# Autodesk Inventor assembly: Spool mount
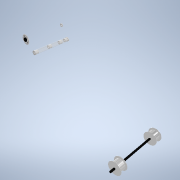
[picture p0: Inventor's stored thumbnail of the model, 180x180]
Saved by Autodesk Inventor 2020 (Build 240168000, 168)
## iProperties
Created: 2020-01-30
Part Number: Spool mount
Document SubType Name: Assembly
Designer: 1cikaychapman
Author: 1cikaychapman
## Documents named in this file (9)
- D:\Users\JimAndVal\Documents\JIM\IronRiders\2020 Robot-1\Climber\Spool mount.iam
- D:\Users\JimAndVal\Documents\JIM\IronRiders\2020 Robot-1\Climber\Hex.ipt
- D:\Users\JimAndVal\Documents\JIM\IronRiders\2020 Robot-1\Climber\Spool.ipt
- D:\Users\JimAndVal\Documents\JIM\IronRiders\2020 Robot-1\Climber\Climber Axel End Cap.ipt
- D:\Users\JimAndVal\Documents\JIM\IronRiders\2020 Robot-1\Climber\Climber Axel Spacer.ipt
- D:\Users\JimAndVal\Documents\JIM\IronRiders\2020 Robot-1\Climber\1 inch sched 40 aluminum pipe - 11 inch long.ipt
- D:\Users\JimAndVal\Documents\JIM\IronRiders\2020 Robot-1\Climber\_34t_Aluminum_Plate_Sprocket_25_Chain_1-1_8_Bearing_Bore_217-2664.ipt
- D:\Users\JimAndVal\Documents\JIM\IronRiders\2020 Robot-1\Climber\1_2_Hex_Bore_Aluminum_VersaHub_217-2592.ipt
- D:\Users\JimAndVal\Documents\JIM\IronRiders\2020 Robot-1\Climber\Clamping_Shaft_Collar_-_1_2_Hex_ID_217-2737(1).ipt
## Components (11 placed, 8 different names)
1. Hex:1 — Mate:1, Mate:2, Mate:3, Mate:4, Flush:1, Flush:2
2. Spool:1 — Mate:1, Mate:2, Flush:2
3. Spool:2 — Mate:3, Mate:4, Flush:1
4. Climber Axel End Cap:1 — Mate:9, Mate:11
5. Climber Axel End Cap:2 — Mate:10
6. Climber Axel Spacer:1 — Mate:7
7. Climber Axel Spacer:2 — Mate:8
8. 1 inch sched 40 aluminum pipe - 11 inch long:1 — Mate:7, Mate:8, Mate:9, Mate:10, Mate:11
9. _34t_Aluminum_Plate_Sprocket_25_Chain_1-1_8_Bearing_Bore_217-2664:1 — Mate:5, Mate:6
10. 1_2_Hex_Bore_Aluminum_VersaHub_217-2592:1 — Mate:5, Mate:6
11. Clamping_Shaft_Collar_-_1_2_Hex_ID_217-2737(1):1
## Relationships (13: Mate 11, Flush 2)
- Mate:1: Hex:1 ↔ Spool:1
- Mate:2: Hex:1 ↔ Spool:1
- Mate:3: Hex:1 ↔ Spool:2
- Mate:4: Hex:1 ↔ Spool:2
- Flush:1 (38.1 mm): Hex:1 ↔ Spool:2
- Flush:2 (38.1 mm): Hex:1 ↔ Spool:1
- Mate:5: _34t_Aluminum_Plate_Sprocket_25_Chain_1-1_8_Bearing_Bore_217-2664:1 ↔ 1_2_Hex_Bore_Aluminum_VersaHub_217-2592:1
- Mate:6: _34t_Aluminum_Plate_Sprocket_25_Chain_1-1_8_Bearing_Bore_217-2664:1 ↔ 1_2_Hex_Bore_Aluminum_VersaHub_217-2592:1
- Mate:7: Climber Axel Spacer:1 ↔ 1 inch sched 40 aluminum pipe - 11 inch long:1
- Mate:8: Climber Axel Spacer:2 ↔ 1 inch sched 40 aluminum pipe - 11 inch long:1
- Mate:9: Climber Axel End Cap:1 ↔ 1 inch sched 40 aluminum pipe - 11 inch long:1
- Mate:10: Climber Axel End Cap:2 ↔ 1 inch sched 40 aluminum pipe - 11 inch long:1
- Mate:11: Climber Axel End Cap:1 ↔ 1 inch sched 40 aluminum pipe - 11 inch long:1
